# Autodesk Inventor assembly: A_beam
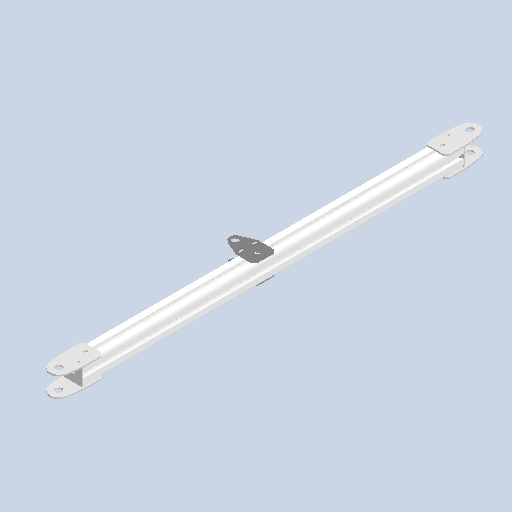
[picture p0: Inventor's stored thumbnail of the model, 512x512]
Saved by Autodesk Inventor 2025.2 (Build 292293000, 293)
## iProperties
Created: 2025-05-02
Part Number: A_beam
Document SubType Name: Assembly
Designer: Caspe
Mass: 2634.61 g
Surface Area: 3263.73 cm^2
Volume: 840.093 cm^3
Density: 3.13609 g/cm^3
Author: Caspe
## Documents named in this file (4)
- C:\Users\Caspe\Documents\Semester 8\Project\Anomaly_Detection\Mechanical_Project\Inventor_project\A_beam.iam
- C:\Users\Caspe\Documents\Semester 8\Project\Anomaly_Detection\Mechanical_Project\Inventor_project\0_0_026_03-1000-Aluflex\0_0_026_03-1000-Aluflex\0_0_026_03-1000-Aluflex.ipt
- C:\Users\Caspe\Documents\Semester 8\Project\Anomaly_Detection\Mechanical_Project\Inventor_project\A_beam_end_mount.iam
- C:\Users\Caspe\Documents\Semester 8\Project\Anomaly_Detection\Mechanical_Project\Inventor_project\A_beam_piston_mount.iam
## Components (4 placed, 3 different names)
1. 0_0_026_03-1000-Aluflex:1 — Mate:3, Mate:4, Mate:5, Mate:6, Mate:7, Mate:8
2. A_beam_end_mount:1 [sub-assembly] — Mate:7, Mate:8
3. A_beam_end_mount:2 [sub-assembly] — Mate:3, Mate:4
4. A_beam_piston_mount:1 [sub-assembly] — Mate:5, Mate:6
## Relationships (6: Mate 6)
- Mate:3: 0_0_026_03-1000-Aluflex:1 ↔ A_beam_end_mount:2
- Mate:4: 0_0_026_03-1000-Aluflex:1 ↔ A_beam_end_mount:2
- Mate:5: 0_0_026_03-1000-Aluflex:1 ↔ A_beam_piston_mount:1
- Mate:6: 0_0_026_03-1000-Aluflex:1 ↔ A_beam_piston_mount:1
- Mate:7: 0_0_026_03-1000-Aluflex:1 ↔ A_beam_end_mount:1
- Mate:8: 0_0_026_03-1000-Aluflex:1 ↔ A_beam_end_mount:1
